# Autodesk Inventor assembly: ASSY.ROLLER
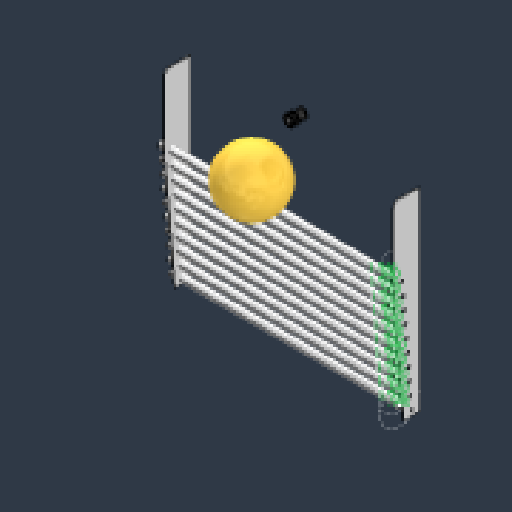
[picture p0: Inventor's stored thumbnail of the model, 512x512]
Saved by Autodesk Inventor 2026 (Build 300175050, 175E)
## iProperties
Created: 2026-04-04
Part Number: ASSY.ROLLER
Document SubType Name: Assembly
Designer: Jthib
Mass: 3428.89 g
Surface Area: 9144.82 cm^2
Volume: 2534.34 cm^3
Density: 1.35297 g/cm^3
Author: Jthib
## Documents named in this file (9)
- C:\Users\Jthib\Documents\GitHub\2026-Robot-Mechanical\Roller\ASSY.ROLLER.iam
- C:\Users\Jthib\Documents\GitHub\2026-Robot-Mechanical\Roller\TUBE,ROLLER,LONG.ipt
- E:\Downloads\WCP-1420\WCP-1420\WCP-1420.ipt
- E:\Downloads\WCP-1803\WCP-1803\WCP-1803.ipt
- C:\Users\Jthib\Documents\GitHub\2026-Robot-Mechanical\#2_2026 Field CAD\GE-26900_ Fuel.ipt
- C:\Users\Jthib\Documents\GitHub\2026-Robot-Mechanical\Roller\PLATE,SIDE.ipt
- C:\Users\Jthib\Documents\GitHub\2026-Robot-Mechanical\Roller\PLATE,SIDE,SHORT.ipt
- C:\Users\Jthib\Documents\GitHub\2026-Robot-Mechanical\Spindexer\3DPRINT,ROLLER,PLUG,SHORT.ipt
- C:\Users\Jthib\Documents\GitHub\2026-Robot-Mechanical\Roller\PLATE,ROLLER,REAR.ipt
## Components (28 placed, 8 different names)
1. WCP-1420:1
2. WCP-1803:1
3. GE-26900_ Fuel:1
4. PLATE,SIDE:1 — Mate:1, Mate:2, Flush:1, Mate:3, Mate:5, Mate:6, Mate:7, Mate:9, Mate:10
5. PLATE,SIDE,SHORT:1 — Flush:2, Flush:3, Mate:4
6. PLATE,ROLLER,REAR:1 — Mate:8, Mate:9, Mate:10
7. 3DPRINT,ROLLER,PLUG,SHORT:9 — Insert:1
8. 3DPRINT,ROLLER,PLUG,SHORT:10 — Insert:3
9. 3DPRINT,ROLLER,PLUG,SHORT:11 — Insert:2
10. TUBE,ROLLER,LONG:5 — Mate:1, Mate:5, Mate:11
11. TUBE,ROLLER,LONG:6
12. TUBE,ROLLER,LONG:7
13. TUBE,ROLLER,LONG:8
14. TUBE,ROLLER,LONG:9
15. TUBE,ROLLER,LONG:10
16. TUBE,ROLLER,LONG:11
17. TUBE,ROLLER,LONG:12
18. TUBE,ROLLER,LONG:13 — Mate:6, Mate:7, Insert:3
19. TUBE,ROLLER,LONG:14 — Insert:2
20. TUBE,ROLLER,LONG:15 — Insert:1
21. 3DPRINT,ROLLER,PLUG,SHORT:1 — Mate:11
22. 3DPRINT,ROLLER,PLUG,SHORT:2
23. 3DPRINT,ROLLER,PLUG,SHORT:3
24. 3DPRINT,ROLLER,PLUG,SHORT:4
25. 3DPRINT,ROLLER,PLUG,SHORT:5
26. 3DPRINT,ROLLER,PLUG,SHORT:6
27. 3DPRINT,ROLLER,PLUG,SHORT:7
28. 3DPRINT,ROLLER,PLUG,SHORT:8
## Component patterns: (8 elements, first: TUBE,ROLLER,LONG:5), (3 elements, first: TUBE,ROLLER,LONG:13), (8 elements, first: 3DPRINT,ROLLER,PLUG,SHORT:1)
## Relationships (17: Mate 11, Flush 3, Insert 3)
- Mate:1: PLATE,SIDE:1 ↔ TUBE,ROLLER,LONG:5
- Mate:2: PLATE,SIDE:1
- Flush:1 (349.25 mm): PLATE,SIDE:1
- Mate:3 (279.4 mm): PLATE,SIDE:1
- Flush:2 (279.4 mm): PLATE,SIDE,SHORT:1
- Flush:3: PLATE,SIDE,SHORT:1
- Mate:4: PLATE,SIDE,SHORT:1
- Mate:5 (3.175 mm): PLATE,SIDE:1 ↔ TUBE,ROLLER,LONG:5
- Mate:6: PLATE,SIDE:1 ↔ TUBE,ROLLER,LONG:13
- Mate:7 (3.175 mm): PLATE,SIDE:1 ↔ TUBE,ROLLER,LONG:13
- Mate:8: PLATE,ROLLER,REAR:1
- Mate:9 (317.5 mm): PLATE,SIDE:1 ↔ PLATE,ROLLER,REAR:1
- Mate:10: PLATE,SIDE:1 ↔ PLATE,ROLLER,REAR:1
- Mate:11: TUBE,ROLLER,LONG:5 ↔ 3DPRINT,ROLLER,PLUG,SHORT:1
- Insert:1: 3DPRINT,ROLLER,PLUG,SHORT:9 ↔ TUBE,ROLLER,LONG:15
- Insert:2: 3DPRINT,ROLLER,PLUG,SHORT:11 ↔ TUBE,ROLLER,LONG:14
- Insert:3: 3DPRINT,ROLLER,PLUG,SHORT:10 ↔ TUBE,ROLLER,LONG:13
